# Autodesk Inventor assembly: thic_thin_comp
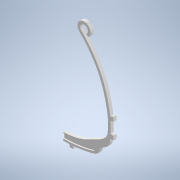
[picture p0: Inventor's stored thumbnail of the model, 180x180]
Saved by Autodesk Inventor 2020 (Build 240168000, 168)
## iProperties
Created: 2020-03-29
Part Number: thic_thin_comp
Document SubType Name: Assembly
Designer: Clevo
Author: Clevo
## Documents named in this file (3)
- E:\Cornell_PPE_InjectionMolding\MaterialPropertiesStudy\thic_thin_comp.iam
- E:\Cornell_PPE_InjectionMolding\headband_IM_ANSYS.ipt
- E:\Cornell_PPE_InjectionMolding\Thicc_headband_IM_ANSYS.ipt
## Components (2 placed, 2 different names)
1. headband_IM_ANSYS:1 — Flush:1, Flush:2, Mate:1
2. Thicc_headband_IM_ANSYS:1 — Flush:1, Flush:2, Mate:1
## Relationships (3: Flush 2, Mate 1)
- Flush:1: headband_IM_ANSYS:1 ↔ Thicc_headband_IM_ANSYS:1
- Flush:2: headband_IM_ANSYS:1 ↔ Thicc_headband_IM_ANSYS:1
- Mate:1: headband_IM_ANSYS:1 ↔ Thicc_headband_IM_ANSYS:1
